# Autodesk Inventor assembly: Lime Extruder - ASM
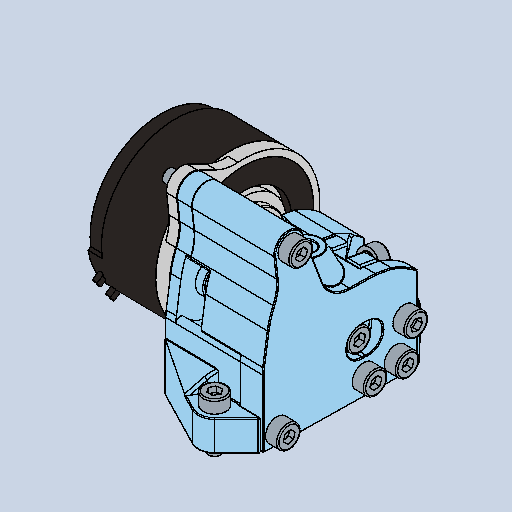
[picture p0: Inventor's stored thumbnail of the model, 512x512]
Saved by Autodesk Inventor 2026 (Build 300175050, 175E)
## iProperties
Created: 2025-07-30
Part Number: Lime Extruder - ASM
Description: STEP AP242
Document SubType Name: Assembly
Designer: tdxt
Sending System: ONSHAPE BY PTC INC, 1.201
Preprocessor: ST-DEVELOPER v20
Title: 688046dff3c7ef29f6bbb4df
## Documents named in this file (9)
- D:\Github\Lime\Lime Extruder - ASM\Lime Extruder - ASM\Lime Extruder - ASM.iam
- D:\Github\Lime\Lime Extruder - ASM\Lime Extruder - ASM\GEAR_7MM_12_TEETH_0_5_3MM_BORE.ipt
- D:\Github\Lime\Lime Extruder - ASM\Lime Extruder - ASM\Hex socket head cap screw M3x0.50 x 20.ipt
- D:\Github\Lime\Lime Extruder - ASM\Lime Extruder - ASM\Hex socket head cap screw M3x0.50 x 10.ipt
- D:\Github\Lime\Lime Extruder - ASM\Lime Extruder - ASM\Idler Arm.ipt
- D:\Github\Lime\Lime Extruder - ASM\Lime Extruder - ASM\Hex socket head cap screw M3x0.50 x 30.ipt
- D:\Github\Lime\Lime Extruder - ASM\Lime Extruder - ASM\Front Frame.ipt
- D:\Github\Lime\Lime Extruder - ASM\Lime Extruder - ASM\K1_EXTRUDER_MOTOR_-_MOONS_CSE14.ipt
- D:\Github\Lime\Lime Extruder - ASM\Lime Extruder - ASM\Back Frame.ipt
## Components (14 placed, 14 different names)
1. NAUO1 — 旋转:1
2. NAUO2 — 旋转:11
3. NAUO3 — 旋转:14
4. NAUO4 — 旋转:6, 旋转:14
5. NAUO5 — 旋转:9
6. NAUO6 — 旋转:2, 旋转:3, 旋转:7, 旋转:9, 旋转:10, 旋转:11, 旋转:12, 旋转:13
7. NAUO7 — 刚性:1
8. NAUO8 — 旋转:12
9. NAUO9 — 旋转:13
10. NAUO10 — 旋转:7
11. NAUO11 — 旋转:1, 旋转:4, 旋转:5
12. NAUO12 — 旋转:8
13. NAUO13 — 旋转:10
14. NAUO14 — 旋转:2, 旋转:3, 旋转:4, 旋转:5, 旋转:6, 刚性:1, 旋转:8
## Relationships (15: RevoluteJoint 14, WeldJoint 1)
- 旋转:1 [RevoluteJoint]: NAUO1 ↔ NAUO11
- 旋转:2 [RevoluteJoint] (-0.1 mm): NAUO6 ↔ NAUO14
- 旋转:3 [RevoluteJoint] (0.2 mm): NAUO6 ↔ NAUO14
- 旋转:4 [RevoluteJoint]: NAUO11 ↔ NAUO14
- 旋转:5 [RevoluteJoint]: NAUO11 ↔ NAUO14
- 旋转:6 [RevoluteJoint] (0.2 mm): NAUO4 ↔ NAUO14
- 旋转:7 [RevoluteJoint] (3 mm): NAUO6 ↔ NAUO10
- 刚性:1 [WeldJoint]: NAUO7 ↔ NAUO14
- 旋转:8 [RevoluteJoint]: NAUO12 ↔ NAUO14
- 旋转:9 [RevoluteJoint]: NAUO5 ↔ NAUO6
- 旋转:10 [RevoluteJoint]: NAUO6 ↔ NAUO13
- 旋转:11 [RevoluteJoint]: NAUO2 ↔ NAUO6
- 旋转:12 [RevoluteJoint]: NAUO6 ↔ NAUO8
- 旋转:13 [RevoluteJoint]: NAUO6 ↔ NAUO9
- 旋转:14 [RevoluteJoint]: NAUO3 ↔ NAUO4
